# Autodesk Inventor assembly: Kitchen.01
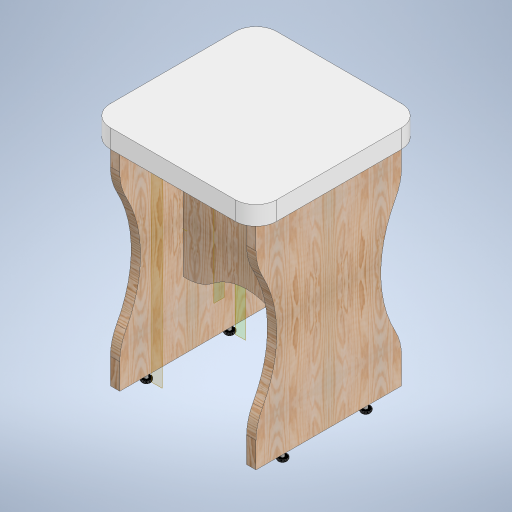
[picture p0: Inventor's stored thumbnail of the model, 512x512]
Saved by Autodesk Inventor 2024 (Build 280153000, 153)
## iProperties
Created: 2016-08-19
Part Number: Kitchen.01
Document SubType Name: Assembly
Designer: SauliusD
Description: Stool
Author: SauliusD
## Documents named in this file (10)
- C:\W4INV 2024 Design\PROJECTS\Samples\Simple Kitchen table and stool\Stool\Stool.iam
- C:\W4INV 2024 Design\PROJECTS\Samples\Simple Kitchen table and stool\Stool\Top.ipt
- C:\W4INV 2024 Design\PROJECTS\Samples\Simple Kitchen table and stool\Stool\Right leg.ipt
- C:\W4INV 2024 Design\PROJECTS\Samples\Simple Kitchen table and stool\Stool\Left leg.ipt
- C:\W4INV 2024 Design\PROJECTS\Samples\Simple Kitchen table and stool\Stool\Confirmation.ipt
- C:\W4INV 2024 Design\_LIBRARY\Fixed joints\Minifix joint\MINIFIX D15 v2\Minifix D15 & Dowel L34 & Cap D15 PB T18 LH.ipt
- C:\W4INV 2024 Design\_LIBRARY\Supports and legs\Supports\ADJUSTABLE SUPPORT\Support M6 H27 D18 with Bushing SB T18.ipt
- C:\W4INV 2024 Design\_LIBRARY\Fixed joints\Minifix joint\MINIFIX D15 v2\Minifix D15 & Dowel L34 & Cap D15 PB T18 RH.ipt
- C:\W4INV 2023 Design\LIBRARY\Fixed joints\Minifix joint\MINIFIX D15 v2.ipt
- C:\W4INV 2023 Design\LIBRARY\Supports and legs\Supports\ADJUSTABLE SUPPORT.ipt
## Components (18 placed, 7 different names)
1. Top:1 — Nestled Board Plane:1, Nestled Board Plane:2, Nestled Board Plane:3, Nestled Board Plane:4, Nestled Board Plane:5, Nestled Board Plane:6
2. Right leg:1 — Pillar Board Side Plane :3, Pillar Board Side Plane :5, Nestled Board Plane:7, Nestled Board Plane:9, Bottom board:1, Side board:2, Bottom board:2, Bottom board:3, Side board:4, Bottom board:4
3. Left leg:1 — Flush:1, Flush:2, Pillar Board Side Plane :4, Pillar Board Side Plane :6, Nestled Board Plane:8, Nestled Board Plane:10, Side board:1, Side board:3
4. Confirmation:1 — Axis Plane:1, Pillar Board Side Plane :1, Axis Plane:2, Pillar Board Side Plane :2, Axis Plane:7, Pillar Board Side Plane :7, Axis Plane:8, Pillar Board Side Plane :8, Axis Plane:9, Pillar Board Side Plane :9, Axis Plane:10, Pillar Board Side Plane :10
5. Minifix D15 & Dowel L34 & Cap D15 PB T18 LH:1 — Axis Plane:1, Nestled Board Plane:1, Pillar Board Side Plane :1
6. Minifix D15 & Dowel L34 & Cap D15 PB T18 RH:2 — Axis Plane:2, Nestled Board Plane:2, Pillar Board Side Plane :2
7. Minifix D15 & Dowel L34 & Cap D15 PB T18 RH:3 — Axis Plane:3, Pillar Board Side Plane :3, Nestled Board Plane:3
8. Minifix D15 & Dowel L34 & Cap D15 PB T18 LH:4 — Axis Plane:4, Pillar Board Side Plane :4, Nestled Board Plane:4
9. Minifix D15 & Dowel L34 & Cap D15 PB T18 LH:5 — Axis Plane:5, Pillar Board Side Plane :5, Nestled Board Plane:5
10. Minifix D15 & Dowel L34 & Cap D15 PB T18 RH:6 — Axis Plane:6, Pillar Board Side Plane :6, Nestled Board Plane:6
11. Minifix D15 & Dowel L34 & Cap D15 PB T18 LH:7 — Axis Plane:7, Nestled Board Plane:7, Pillar Board Side Plane :7
12. Minifix D15 & Dowel L34 & Cap D15 PB T18 RH:8 — Axis Plane:8, Nestled Board Plane:8, Pillar Board Side Plane :8
13. Minifix D15 & Dowel L34 & Cap D15 PB T18 RH:9 — Axis Plane:9, Nestled Board Plane:9, Pillar Board Side Plane :9
14. Minifix D15 & Dowel L34 & Cap D15 PB T18 LH:10 — Axis Plane:10, Nestled Board Plane:10, Pillar Board Side Plane :10
15. Support M6 H27 D18 with Bushing SB T18:1 — Axis:1, Side board:1, Bottom board:1
16. Support M6 H27 D18 with Bushing SB T18:2 — Axis:2, Side board:2, Bottom board:2
17. Support M6 H27 D18 with Bushing SB T18:3 — Axis:3, Side board:3, Bottom board:3
18. Support M6 H27 D18 with Bushing SB T18:4 — Axis:4, Side board:4, Bottom board:4
## Relationships (44: Mate 28, Flush 16)
- Flush:1 (-60 mm): Left leg:1
- Flush:2 (-60 mm): Left leg:1
- Axis Plane:1 [Mate]: Confirmation:1 ↔ Minifix D15 & Dowel L34 & Cap D15 PB T18 LH:1
- Nestled Board Plane:1 [Mate]: Top:1 ↔ Minifix D15 & Dowel L34 & Cap D15 PB T18 LH:1
- Pillar Board Side Plane :1 [Flush] (18 mm): Confirmation:1 ↔ Minifix D15 & Dowel L34 & Cap D15 PB T18 LH:1
- Axis Plane:2 [Mate]: Confirmation:1 ↔ Minifix D15 & Dowel L34 & Cap D15 PB T18 RH:2
- Nestled Board Plane:2 [Mate]: Top:1 ↔ Minifix D15 & Dowel L34 & Cap D15 PB T18 RH:2
- Pillar Board Side Plane :2 [Flush] (18 mm): Confirmation:1 ↔ Minifix D15 & Dowel L34 & Cap D15 PB T18 RH:2
- Axis Plane:3 [Mate]: Minifix D15 & Dowel L34 & Cap D15 PB T18 RH:3
- Pillar Board Side Plane :3 [Flush] (18 mm): Right leg:1 ↔ Minifix D15 & Dowel L34 & Cap D15 PB T18 RH:3
- Nestled Board Plane:3 [Mate]: Top:1 ↔ Minifix D15 & Dowel L34 & Cap D15 PB T18 RH:3
- Axis Plane:4 [Mate]: Minifix D15 & Dowel L34 & Cap D15 PB T18 LH:4
- Pillar Board Side Plane :4 [Flush] (18 mm): Left leg:1 ↔ Minifix D15 & Dowel L34 & Cap D15 PB T18 LH:4
- Nestled Board Plane:4 [Mate]: Top:1 ↔ Minifix D15 & Dowel L34 & Cap D15 PB T18 LH:4
- Axis Plane:5 [Mate]: Minifix D15 & Dowel L34 & Cap D15 PB T18 LH:5
- Pillar Board Side Plane :5 [Flush] (18 mm): Right leg:1 ↔ Minifix D15 & Dowel L34 & Cap D15 PB T18 LH:5
- Nestled Board Plane:5 [Mate]: Top:1 ↔ Minifix D15 & Dowel L34 & Cap D15 PB T18 LH:5
- Axis Plane:6 [Mate]: Minifix D15 & Dowel L34 & Cap D15 PB T18 RH:6
- Pillar Board Side Plane :6 [Flush] (18 mm): Left leg:1 ↔ Minifix D15 & Dowel L34 & Cap D15 PB T18 RH:6
- Nestled Board Plane:6 [Mate]: Top:1 ↔ Minifix D15 & Dowel L34 & Cap D15 PB T18 RH:6
- Axis Plane:7 [Mate]: Confirmation:1 ↔ Minifix D15 & Dowel L34 & Cap D15 PB T18 LH:7
- Nestled Board Plane:7 [Mate]: Right leg:1 ↔ Minifix D15 & Dowel L34 & Cap D15 PB T18 LH:7
- Pillar Board Side Plane :7 [Flush] (18 mm): Confirmation:1 ↔ Minifix D15 & Dowel L34 & Cap D15 PB T18 LH:7
- Axis Plane:8 [Mate]: Confirmation:1 ↔ Minifix D15 & Dowel L34 & Cap D15 PB T18 RH:8
- Nestled Board Plane:8 [Mate]: Left leg:1 ↔ Minifix D15 & Dowel L34 & Cap D15 PB T18 RH:8
- Pillar Board Side Plane :8 [Flush] (18 mm): Confirmation:1 ↔ Minifix D15 & Dowel L34 & Cap D15 PB T18 RH:8
- Axis Plane:9 [Mate]: Confirmation:1 ↔ Minifix D15 & Dowel L34 & Cap D15 PB T18 RH:9
- Nestled Board Plane:9 [Mate]: Right leg:1 ↔ Minifix D15 & Dowel L34 & Cap D15 PB T18 RH:9
- Pillar Board Side Plane :9 [Flush] (18 mm): Confirmation:1 ↔ Minifix D15 & Dowel L34 & Cap D15 PB T18 RH:9
- Axis Plane:10 [Mate]: Confirmation:1 ↔ Minifix D15 & Dowel L34 & Cap D15 PB T18 LH:10
- Nestled Board Plane:10 [Mate]: Left leg:1 ↔ Minifix D15 & Dowel L34 & Cap D15 PB T18 LH:10
- Pillar Board Side Plane :10 [Flush] (18 mm): Confirmation:1 ↔ Minifix D15 & Dowel L34 & Cap D15 PB T18 LH:10
- Axis:1 [Mate]: Support M6 H27 D18 with Bushing SB T18:1
- Side board:1 [Flush] (9 mm): Left leg:1 ↔ Support M6 H27 D18 with Bushing SB T18:1
- Bottom board:1 [Mate] (17.5 mm): Right leg:1 ↔ Support M6 H27 D18 with Bushing SB T18:1
- Axis:2 [Mate]: Support M6 H27 D18 with Bushing SB T18:2
- Side board:2 [Flush] (9 mm): Right leg:1 ↔ Support M6 H27 D18 with Bushing SB T18:2
- Bottom board:2 [Mate] (17.5 mm): Right leg:1 ↔ Support M6 H27 D18 with Bushing SB T18:2
- Axis:3 [Mate]: Support M6 H27 D18 with Bushing SB T18:3
- Side board:3 [Flush] (9 mm): Left leg:1 ↔ Support M6 H27 D18 with Bushing SB T18:3
- Bottom board:3 [Mate] (17.5 mm): Right leg:1 ↔ Support M6 H27 D18 with Bushing SB T18:3
- Axis:4 [Mate]: Support M6 H27 D18 with Bushing SB T18:4
- Side board:4 [Flush] (9 mm): Right leg:1 ↔ Support M6 H27 D18 with Bushing SB T18:4
- Bottom board:4 [Mate] (17.5 mm): Right leg:1 ↔ Support M6 H27 D18 with Bushing SB T18:4
